# Autodesk Inventor assembly: Assembly of Cover+Plate+Event Camera
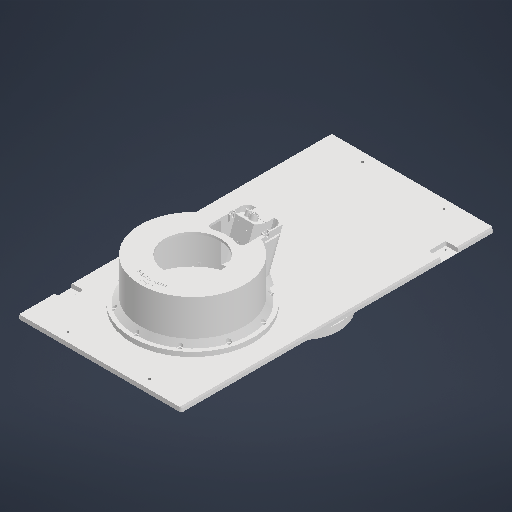
[picture p0: Inventor's stored thumbnail of the model, 512x512]
Saved by Autodesk Inventor 2027 (Build 310192000, 192)
## iProperties
Created: 2026-01-19
Part Number: Assembly of Cover+Plate+Event Camera
Document SubType Name: Assembly
Designer: AdminForWorker
Title: Assembly of Cover+Plate+Event Camera v6
Author: AdminForWorker
## Documents named in this file (8)
- C:\Users\ig2\Desktop\Branding\LPBF-Observer\system_development\Turin\v0.4\Assembly\Assembly of Cover+Plate+Event Camera.iam
- C:\Users\ig2\Desktop\Branding\LPBF-Observer\system_development\Turin\v0.4\Assembly\Build Plate v1.ipt
- C:\Users\ig2\Desktop\Branding\LPBF-Observer\system_development\Turin\v0.4\Assembly\Triton2_Imported v1.ipt
- C:\Users\ig2\Desktop\Branding\LPBF-Observer\system_development\Turin\v0.4\Assembly\M3 35 mm 18-8 Stainless Steel Socket Head Screw.ipt
- C:\Users\ig2\Desktop\Branding\LPBF-Observer\system_development\Turin\v0.4\Assembly\M3 316 Stainless Steel Hex Nut.ipt
- C:\Users\ig2\Desktop\Branding\LPBF-Observer\system_development\Turin\v0.4\Assembly\12mm Turin Cover.ipt
- C:\Users\ig2\Desktop\Branding\LPBF-Observer\system_development\Turin\v0.4\Assembly\316 Stainless Steel General Purpose Washer.ipt
- C:\Users\ig2\Desktop\Branding\LPBF-Observer\system_development\Turin\v0.4\Assembly\Turin Camera Cylinder Housing.ipt
## Components (13 placed, 7 different names)
1. M3 316 Stainless Steel Hex Nut:5
2. Triton2_Imported v1:1 — Rotational:11
3. M3 35 mm 18-8 Stainless Steel Socket Head Screw:1 — Rotational:19
4. M3 35 mm 18-8 Stainless Steel Socket Head Screw:2 — Rotational:17
5. M3 35 mm 18-8 Stainless Steel Socket Head Screw:3 — Rotational:16
6. M3 35 mm 18-8 Stainless Steel Socket Head Screw:4 — Rotational:18
7. Build Plate v1:1
8. Turin Camera Cylinder Housing:1 — Rotational:10, Rotational:11, Rotational:12, Rotational:13, Rotational:14, Rotational:15
9. 12mm Turin Cover:1 — Rotational:10
10. 316 Stainless Steel General Purpose Washer:5 — Rotational:15, Rotational:19
11. 316 Stainless Steel General Purpose Washer:6 — Rotational:13, Rotational:17
12. 316 Stainless Steel General Purpose Washer:7 — Rotational:14, Rotational:18
13. 316 Stainless Steel General Purpose Washer:8 — Rotational:12, Rotational:16
## Relationships (10: RevoluteJoint 10)
- Rotational:10 [RevoluteJoint]: Turin Camera Cylinder Housing:1 ↔ 12mm Turin Cover:1
- Rotational:11 [RevoluteJoint]: Triton2_Imported v1:1 ↔ Turin Camera Cylinder Housing:1
- Rotational:12 [RevoluteJoint]: Turin Camera Cylinder Housing:1 ↔ 316 Stainless Steel General Purpose Washer:8
- Rotational:13 [RevoluteJoint]: Turin Camera Cylinder Housing:1 ↔ 316 Stainless Steel General Purpose Washer:6
- Rotational:14 [RevoluteJoint]: Turin Camera Cylinder Housing:1 ↔ 316 Stainless Steel General Purpose Washer:7
- Rotational:15 [RevoluteJoint]: Turin Camera Cylinder Housing:1 ↔ 316 Stainless Steel General Purpose Washer:5
- Rotational:16 [RevoluteJoint]: M3 35 mm 18-8 Stainless Steel Socket Head Screw:3 ↔ 316 Stainless Steel General Purpose Washer:8
- Rotational:17 [RevoluteJoint]: M3 35 mm 18-8 Stainless Steel Socket Head Screw:2 ↔ 316 Stainless Steel General Purpose Washer:6
- Rotational:18 [RevoluteJoint]: M3 35 mm 18-8 Stainless Steel Socket Head Screw:4 ↔ 316 Stainless Steel General Purpose Washer:7
- Rotational:19 [RevoluteJoint]: M3 35 mm 18-8 Stainless Steel Socket Head Screw:1 ↔ 316 Stainless Steel General Purpose Washer:5
